# Autodesk Inventor assembly: 19K_001_010_00_A_RIM_10_2019_EFRE_3D
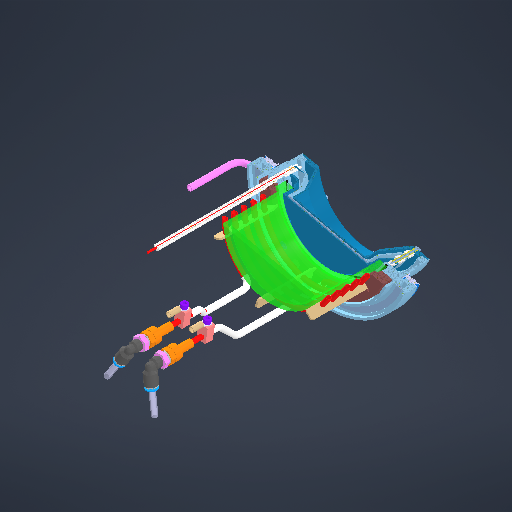
[picture p0: Inventor's stored thumbnail of the model, 512x512]
Saved by Autodesk Inventor 2027 (Build 310192060, 192F)
## iProperties
Company: none
Created: 2025-10-08
Part Number: 19K_001_010_00_A_RIM_10_2019_EFRE_3D
Description: CATIA V5 STEP
Document SubType Name: Assembly
Designer: kw
Authority: none
Title: 19K_001_010_00_A_RIM_10_2019_EFRE_3D_2024_0228.stp
Author: Halle20
Revision Number: A
Sending System: Autodesk Inventor 2024
Preprocessor: ST-DEVELOPER v20
## Documents named in this file (6)
- C:\Users\kw\OneDrive\Documents\Uni\Masterthesis\Spezialisierungsmodul\InventorZeichnungen\19K_001_010_00_A_RIM_10_2019_EFRE_3D_2024_0228\19K_001_010_00_A_RIM_10_2019_EFRE_3D_2024_0228.iam
- C:\Users\kw\OneDrive\Documents\Uni\Masterthesis\Spezialisierungsmodul\InventorZeichnungen\19K_001_010_00_A_RIM_10_2019_EFRE_3D_2024_0228\15K_019_028_00_A_HF_VERSORGUNG.iam
- C:\Users\kw\OneDrive\Documents\Uni\Masterthesis\Spezialisierungsmodul\InventorZeichnungen\19K_001_010_00_A_RIM_10_2019_EFRE_3D_2024_0228\15P_019_030_00_A_TOEPFE_MIT_GITTER_3D.iam
- C:\Users\kw\OneDrive\Documents\Uni\Masterthesis\Spezialisierungsmodul\InventorZeichnungen\19K_001_010_00_A_RIM_10_2019_EFRE_3D_2024_0228\15K_019_010_00_A_80XX_00_ISO_K_ZENTRIERRING_AUSSEN_312 ZRA 160.ipt
- C:\Users\kw\OneDrive\Documents\Uni\Masterthesis\Spezialisierungsmodul\InventorZeichnungen\19K_001_010_00_A_RIM_10_2019_EFRE_3D_2024_0228\15K_019_025_00_A_GRUNDTRAEGER_ISO_K_160_OPTI_3D.iam
- C:\Users\kw\OneDrive\Documents\Uni\Masterthesis\Spezialisierungsmodul\InventorZeichnungen\19K_001_010_00_A_RIM_10_2019_EFRE_3D_2024_0228\19K_001_040_00_A_GEFAESS_SPULE_3D.iam
## Components (5 placed, 5 different names)
1. 15K_019_028_00_A_HF_VERSORGUNG.1 [sub-assembly] — Mate:6, Mate:9, Mate:11
2. 15P_019_030_00_A_TOEPFE_MIT_GITTER_3D.1 [sub-assembly] — Mate:3, Mate:4, Mate:5, Mate:6, Mate:11
3. 15K_019_010_00_A_80XX_00_ISO_K_ZENTRIERRING_AUSSEN_312 ZRA 160.1 — Mate:1, Mate:2
4. 15K_019_025_00_A_GRUNDTRAEGER_ISO_K_160_OPTI_3D.1 [sub-assembly] — Mate:1, Mate:2, Mate:3, Mate:4, Mate:5, Mate:7, Mate:8, Mate:10
5. 19K_001_040_00_A_GEFAESS_SPULE_3D.1 [sub-assembly] — Mate:7, Mate:8, Mate:9, Mate:10
## Relationships (11: Mate 11)
- Mate:1: 15K_019_010_00_A_80XX_00_ISO_K_ZENTRIERRING_AUSSEN_312 ZRA 160.1 ↔ 15K_019_025_00_A_GRUNDTRAEGER_ISO_K_160_OPTI_3D.1
- Mate:2: 15K_019_010_00_A_80XX_00_ISO_K_ZENTRIERRING_AUSSEN_312 ZRA 160.1 ↔ 15K_019_025_00_A_GRUNDTRAEGER_ISO_K_160_OPTI_3D.1
- Mate:3: 15P_019_030_00_A_TOEPFE_MIT_GITTER_3D.1 ↔ 15K_019_025_00_A_GRUNDTRAEGER_ISO_K_160_OPTI_3D.1
- Mate:4: 15P_019_030_00_A_TOEPFE_MIT_GITTER_3D.1 ↔ 15K_019_025_00_A_GRUNDTRAEGER_ISO_K_160_OPTI_3D.1
- Mate:5: 15P_019_030_00_A_TOEPFE_MIT_GITTER_3D.1 ↔ 15K_019_025_00_A_GRUNDTRAEGER_ISO_K_160_OPTI_3D.1
- Mate:6: 15K_019_028_00_A_HF_VERSORGUNG.1 ↔ 15P_019_030_00_A_TOEPFE_MIT_GITTER_3D.1
- Mate:7: 15K_019_025_00_A_GRUNDTRAEGER_ISO_K_160_OPTI_3D.1 ↔ 19K_001_040_00_A_GEFAESS_SPULE_3D.1
- Mate:8: 15K_019_025_00_A_GRUNDTRAEGER_ISO_K_160_OPTI_3D.1 ↔ 19K_001_040_00_A_GEFAESS_SPULE_3D.1
- Mate:9: 15K_019_028_00_A_HF_VERSORGUNG.1 ↔ 19K_001_040_00_A_GEFAESS_SPULE_3D.1
- Mate:10: 15K_019_025_00_A_GRUNDTRAEGER_ISO_K_160_OPTI_3D.1 ↔ 19K_001_040_00_A_GEFAESS_SPULE_3D.1
- Mate:11: 15K_019_028_00_A_HF_VERSORGUNG.1 ↔ 15P_019_030_00_A_TOEPFE_MIT_GITTER_3D.1
